# Autodesk Inventor assembly: shooter
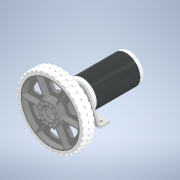
[picture p0: Inventor's stored thumbnail of the model, 180x180]
Saved by Autodesk Inventor 2020.2 (Build 242310000, 310)
## iProperties
Created: 2020-01-12
Part Number: shooter
Document SubType Name: Assembly
Designer: robst
Author: robst
## Documents named in this file (5)
- C:\git\CAD-Development\robSteele\2020CompetitionRobot\shooter.iam
- C:\git\CAD-Development\robSteele\2020LongRobotBase\am-0255 2.5inch CIM Motor.ipt
- C:\git\CAD-Development\robSteele\2020LongRobotBase\6 HiGrip Asm Rev II.iam
- C:\git\CAD-Development\robSteele\2020LongRobotBase\AM 2488 CIM bracket.ipt
- C:\git\CAD-Development\robSteele\2020LongRobotBase\am-0320a_8mm_Key_Hub.ipt
## Components (4 placed, 4 different names)
1. am-0255 2.5inch CIM Motor:1 — Insert:1, Insert:2, Insert:3
2. 6 HiGrip Asm Rev II:1 [sub-assembly] — Insert:4, Mate:1
3. AM 2488 CIM bracket:1 — Insert:1, Insert:2, Angle:1
4. am-0320a_8mm_Key_Hub:1 — Insert:3, Insert:4
## Relationships (6: Insert 4, Mate 1, Angle 1)
- Insert:1: am-0255 2.5inch CIM Motor:1 ↔ AM 2488 CIM bracket:1
- Insert:2: am-0255 2.5inch CIM Motor:1 ↔ AM 2488 CIM bracket:1
- Insert:3: am-0255 2.5inch CIM Motor:1 ↔ am-0320a_8mm_Key_Hub:1
- Insert:4: 6 HiGrip Asm Rev II:1 ↔ am-0320a_8mm_Key_Hub:1
- Mate:1: 6 HiGrip Asm Rev II:1
- Angle:1 (0 deg): AM 2488 CIM bracket:1
